# Autodesk Inventor assembly: CIM for Single Stage Vex Box
Saved by Autodesk Inventor 2013 (Build 170138000, 138)
## iProperties
Created: 2013-01-06
Part Number: CIM for Single Stage Vex Box
Document SubType Name: Assembly
Designer: Nemo
Author: Nemo
## Documents named in this file (4)
- H:\Nemo\Documents\Robotics\VexPro\Gearbox - Single Reduction\CIM for Single Stage Vex Box.iam
- H:\Nemo\Documents\Robotics\COTS Parts\Motors\CIM motor.ipt
- H:\Nemo\Documents\Robotics\COTS Parts\Fasteners\10-32 SHCS x625.ipt
- H:\Nemo\Documents\Robotics\VexPro\Gears\Gear 20dp 10mm key 12T Vex.ipt
## Components (4 placed, 3 different names)
1. CIM motor:1
2. 10-32 SHCS x625:1
3. 10-32 SHCS x625:2
4. Gear 20dp 10mm key 12T Vex:1
## Relationships (5: Insert 2, Mate 2, Angle 1)
- [Insert] (3.175 mm): CIM motor:1 ↔ 10-32 SHCS x625:1
- [Insert] (3.175 mm): CIM motor:1 ↔ 10-32 SHCS x625:2
- [Mate]: CIM motor:1 ↔ Gear 20dp 10mm key 12T Vex:1
- [Angle] (0 deg): CIM motor:1 ↔ Gear 20dp 10mm key 12T Vex:1
- [Mate] (3.175 mm): CIM motor:1 ↔ Gear 20dp 10mm key 12T Vex:1
